# Autodesk Inventor assembly: Attacker_v1
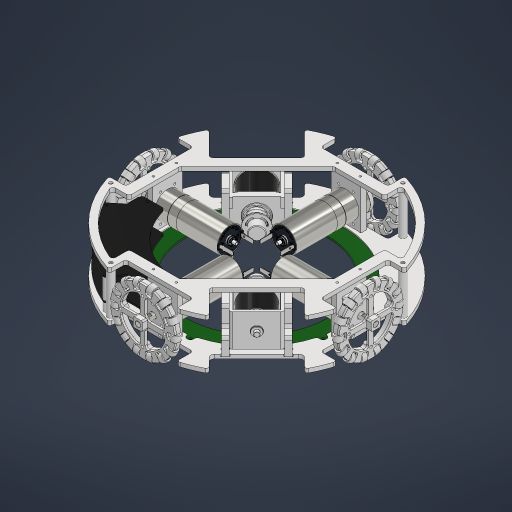
[picture p0: Inventor's stored thumbnail of the model, 512x512]
Saved by Autodesk Inventor 2024.2 (Build 282272000, 272)
## iProperties
Created: 2023-12-21
Part Number: Attacker_v1
Document SubType Name: Assembly
Designer: Hanaoka
Author: Hanaoka
## Documents named in this file (12)
- G:\共有ドライブ\reRo\05_個人\hanaoka\inventor\Attacker_v1.iam
- G:\共有ドライブ\reRo\05_個人\hanaoka\inventor\DriveUnit.iam
- G:\共有ドライブ\reRo\05_個人\hanaoka\inventor\BasePlate.ipt
- G:\共有ドライブ\reRo\05_個人\hanaoka\inventor\Spacer_M2.6x35.ipt
- G:\共有ドライブ\reRo\05_個人\hanaoka\inventor\Ball.ipt
- G:\共有ドライブ\reRo\05_個人\hanaoka\inventor\LineSensor_PCB.ipt
- G:\共有ドライブ\reRo\05_個人\hanaoka\inventor\Spacer_M2x8.ipt
- G:\共有ドライブ\reRo\05_個人\hanaoka\inventor\MainMCU_PCB.ipt
- G:\共有ドライブ\reRo\05_個人\hanaoka\inventor\Spacer_M2x15.ipt
- G:\共有ドライブ\reRo\05_個人\hanaoka\inventor\MotorDriver_PCB.ipt
- G:\共有ドライブ\reRo\05_個人\hanaoka\inventor\KickerUnit.iam
- G:\共有ドライブ\reRo\05_個人\hanaoka\inventor\SecondPlate.ipt
## Components (24 placed, 11 different names)
1. BasePlate:1 — メイト:1, メイト:2, メイト:3, メイト:4, 挿入:1, メイト:5, メイト:6, メイト:7, メイト:8, メイト:9, メイト:10, メイト:11, メイト:12, メイト:13, メイト:14, メイト:15, メイト:16, 挿入:2, 挿入:3, 挿入:4, フラッシュ:1, フラッシュ:2, 挿入:5, 挿入:6, 挿入:7, 挿入:8, メイト:25, メイト:26, メイト:27, メイト:28, メイト:29, メイト:30
2. DriveUnit:1 [sub-assembly] — メイト:2, メイト:3, メイト:4
3. DriveUnit:2 [sub-assembly] — メイト:7, メイト:10, メイト:11
4. DriveUnit:3 [sub-assembly] — メイト:6, メイト:8, メイト:9
5. DriveUnit:4 [sub-assembly] — メイト:5, メイト:12, メイト:13
6. Spacer_M2.6x35:1 — 挿入:1
7. Spacer_M2.6x35:2 — メイト:16, 挿入:3, フラッシュ:5
8. Spacer_M2.6x35:3 — メイト:15, 挿入:4
9. Spacer_M2.6x35:4 — メイト:14, 挿入:2
10. Ball:1
11. LineSensor_PCB:1 — フラッシュ:1, フラッシュ:2
12. Spacer_M2x8:1 — 挿入:5, フラッシュ:3
13. Spacer_M2x8:2 — 挿入:6
14. Spacer_M2x8:3 — 挿入:7
15. Spacer_M2x8:4 — 挿入:8
16. MainMCU_PCB:1 — フラッシュ:3
17. Spacer_M2x15:2
18. Spacer_M2x15:3
19. Spacer_M2x15:4 — フラッシュ:4
20. Spacer_M2x15:1
21. MotorDriver_PCB:1 — フラッシュ:4
22. KickerUnit:1 [sub-assembly] — メイト:25, メイト:26, メイト:27
23. KickerUnit:2 [sub-assembly] — メイト:28, メイト:29, メイト:30
24. SecondPlate:1 — フラッシュ:5
## Relationships (43: Mate 30, Insert 8, Flush 5)
- メイト:1 [Mate]: BasePlate:1
- メイト:2 [Mate]: BasePlate:1 ↔ DriveUnit:1
- メイト:3 [Mate]: BasePlate:1 ↔ DriveUnit:1
- メイト:4 [Mate]: BasePlate:1 ↔ DriveUnit:1
- 挿入:1 [Insert]: BasePlate:1 ↔ Spacer_M2.6x35:1
- メイト:5 [Mate]: BasePlate:1 ↔ DriveUnit:4
- メイト:6 [Mate]: BasePlate:1 ↔ DriveUnit:3
- メイト:7 [Mate]: BasePlate:1 ↔ DriveUnit:2
- メイト:8 [Mate]: BasePlate:1 ↔ DriveUnit:3
- メイト:9 [Mate]: BasePlate:1 ↔ DriveUnit:3
- メイト:10 [Mate]: BasePlate:1 ↔ DriveUnit:2
- メイト:11 [Mate]: BasePlate:1 ↔ DriveUnit:2
- メイト:12 [Mate]: BasePlate:1 ↔ DriveUnit:4
- メイト:13 [Mate]: BasePlate:1 ↔ DriveUnit:4
- メイト:14 [Mate]: BasePlate:1 ↔ Spacer_M2.6x35:4
- メイト:15 [Mate]: BasePlate:1 ↔ Spacer_M2.6x35:3
- メイト:16 [Mate]: BasePlate:1 ↔ Spacer_M2.6x35:2
- 挿入:2 [Insert]: BasePlate:1 ↔ Spacer_M2.6x35:4
- 挿入:3 [Insert]: BasePlate:1 ↔ Spacer_M2.6x35:2
- 挿入:4 [Insert]: BasePlate:1 ↔ Spacer_M2.6x35:3
- フラッシュ:1 [Flush]: BasePlate:1 ↔ LineSensor_PCB:1
- フラッシュ:2 [Flush]: BasePlate:1 ↔ LineSensor_PCB:1
- 挿入:5 [Insert]: BasePlate:1 ↔ Spacer_M2x8:1
- 挿入:6 [Insert]: BasePlate:1 ↔ Spacer_M2x8:2
- 挿入:7 [Insert]: BasePlate:1 ↔ Spacer_M2x8:3
- 挿入:8 [Insert]: BasePlate:1 ↔ Spacer_M2x8:4
- フラッシュ:3 [Flush]: Spacer_M2x8:1 ↔ MainMCU_PCB:1
- [Mate]: MainMCU_PCB:1 ↔ Spacer_M2x15:3
- [Mate]: MainMCU_PCB:1 ↔ Spacer_M2x15:4
- [Mate]: MainMCU_PCB:1 ↔ Spacer_M2x15:1
- [Mate]: MainMCU_PCB:1 ↔ Spacer_M2x15:2
- [Mate]: MainMCU_PCB:1 ↔ Spacer_M2x15:1
- [Mate]: MainMCU_PCB:1 ↔ Spacer_M2x15:2
- [Mate]: MainMCU_PCB:1 ↔ Spacer_M2x15:3
- [Mate]: MainMCU_PCB:1 ↔ Spacer_M2x15:4
- フラッシュ:4 [Flush]: Spacer_M2x15:4 ↔ MotorDriver_PCB:1
- メイト:25 [Mate]: BasePlate:1 ↔ KickerUnit:1
- メイト:26 [Mate]: BasePlate:1 ↔ KickerUnit:1
- メイト:27 [Mate]: BasePlate:1 ↔ KickerUnit:1
- メイト:28 [Mate]: BasePlate:1 ↔ KickerUnit:2
- メイト:29 [Mate]: BasePlate:1 ↔ KickerUnit:2
- メイト:30 [Mate]: BasePlate:1 ↔ KickerUnit:2
- フラッシュ:5 [Flush]: Spacer_M2.6x35:2 ↔ SecondPlate:1
